# Autodesk Inventor assembly: MisumiLeft
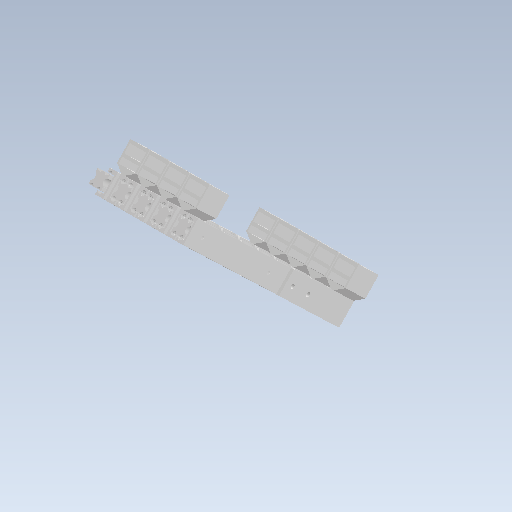
[picture p0: Inventor's stored thumbnail of the model, 512x512]
Saved by Autodesk Inventor 2020 (Build 240168000, 168)
## iProperties
Created: 2020-01-13
Part Number: MisumiLeft
Document SubType Name: Assembly
Designer: tdmp4
Author: tdmp4
## Documents named in this file (3)
- C:\Users\tdmp4\OneDrive\Documents\GitHub\CAD-2020\Misumi\MisumiLeft.iam
- C:\Users\tdmp4\OneDrive\Documents\GitHub\CAD-2020\Misumi\SAR320.iam
- C:\Users\tdmp4\OneDrive\Documents\GitHub\CAD-2020\Misumi\VbearingBracket.ipt
## Components (14 placed, 2 different names)
1. SAR320:1 [sub-assembly] — Mate:1, Mate:2, Flush:1, Mate:3, Mate:4, Flush:2, Flush:13
2. SAR320:2 [sub-assembly] — Mate:5, Mate:6, Mate:7, Mate:8, Mate:9, Flush:3, Mate:11, Mate:12, Flush:4, Flush:13, Flush:14, Flush:18
3. VbearingBracket:1 — Mate:1, Mate:2, Flush:1, Mate:5, Mate:7
4. VbearingBracket:2 — Mate:3, Mate:4, Flush:2, Mate:6
5. VbearingBracket:3 — Mate:8, Mate:9, Flush:3
6. VbearingBracket:4 — Mate:11, Mate:12, Flush:4, Mate:13, Mate:14, Flush:5
7. VbearingBracket:5 — Mate:21, Mate:22, Flush:7
8. VbearingBracket:6 — Mate:27, Mate:28, Flush:10, Flush:11
9. VbearingBracket:7 — Mate:15, Mate:16, Flush:6, Mate:23, Mate:24, Flush:8
10. VbearingBracket:8 — Mate:25, Mate:26, Flush:9, Mate:29, Mate:30
11. SAR320:3 [sub-assembly] — Mate:13, Mate:14, Flush:5, Mate:15, Mate:16, Flush:6, Mate:21, Mate:22, Flush:7, Flush:14, Flush:17, Flush:19
12. SAR320:5 [sub-assembly] — Mate:23, Mate:24, Flush:8, Mate:25, Mate:26, Flush:9, Mate:27, Mate:28, Flush:10, Flush:15, Flush:16, Flush:19, Flush:20
13. SAR320:6 [sub-assembly] — Mate:29, Mate:30, Flush:11, Mate:31, Mate:32, Flush:12, Flush:15, Flush:16, Flush:17, Flush:18, Flush:20
14. VbearingBracket:10 — Mate:31, Mate:32, Flush:12
## Relationships (47: Mate 27, Flush 20)
- Mate:1: SAR320:1 ↔ VbearingBracket:1
- Mate:2: SAR320:1 ↔ VbearingBracket:1
- Flush:1: SAR320:1 ↔ VbearingBracket:1
- Mate:3: SAR320:1 ↔ VbearingBracket:2
- Mate:4: SAR320:1 ↔ VbearingBracket:2
- Flush:2: SAR320:1 ↔ VbearingBracket:2
- Mate:5: SAR320:2 ↔ VbearingBracket:1
- Mate:6: SAR320:2 ↔ VbearingBracket:2
- Mate:7: SAR320:2 ↔ VbearingBracket:1
- Mate:8: SAR320:2 ↔ VbearingBracket:3
- Mate:9: SAR320:2 ↔ VbearingBracket:3
- Flush:3: SAR320:2 ↔ VbearingBracket:3
- Mate:11: SAR320:2 ↔ VbearingBracket:4
- Mate:12: SAR320:2 ↔ VbearingBracket:4
- Flush:4: SAR320:2 ↔ VbearingBracket:4
- Mate:13: VbearingBracket:4 ↔ SAR320:3
- Mate:14: VbearingBracket:4 ↔ SAR320:3
- Flush:5: VbearingBracket:4 ↔ SAR320:3
- Mate:15: VbearingBracket:7 ↔ SAR320:3
- Mate:16: VbearingBracket:7 ↔ SAR320:3
- Flush:6: VbearingBracket:7 ↔ SAR320:3
- Mate:21: VbearingBracket:5 ↔ SAR320:3
- Mate:22: VbearingBracket:5 ↔ SAR320:3
- Flush:7: VbearingBracket:5 ↔ SAR320:3
- Mate:23: VbearingBracket:7 ↔ SAR320:5
- Mate:24: VbearingBracket:7 ↔ SAR320:5
- Flush:8: VbearingBracket:7 ↔ SAR320:5
- Mate:25: VbearingBracket:8 ↔ SAR320:5
- Mate:26: VbearingBracket:8 ↔ SAR320:5
- Flush:9: VbearingBracket:8 ↔ SAR320:5
- Mate:27: VbearingBracket:6 ↔ SAR320:5
- Mate:28: VbearingBracket:6 ↔ SAR320:5
- Flush:10: VbearingBracket:6 ↔ SAR320:5
- Mate:29: VbearingBracket:8 ↔ SAR320:6
- Mate:30: VbearingBracket:8 ↔ SAR320:6
- Flush:11: VbearingBracket:6 ↔ SAR320:6
- Mate:31: SAR320:6 ↔ VbearingBracket:10
- Mate:32: SAR320:6 ↔ VbearingBracket:10
- Flush:12: SAR320:6 ↔ VbearingBracket:10
- Flush:13: SAR320:1 ↔ SAR320:2
- Flush:14: SAR320:2 ↔ SAR320:3
- Flush:15: SAR320:5 ↔ SAR320:6
- Flush:16: SAR320:5 ↔ SAR320:6
- Flush:17: SAR320:3 ↔ SAR320:6
- Flush:18: SAR320:2 ↔ SAR320:6
- Flush:19: SAR320:3 ↔ SAR320:5
- Flush:20: SAR320:5 ↔ SAR320:6
